# Autodesk Inventor assembly: 垃圾桶
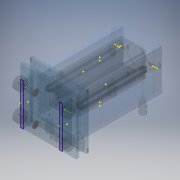
[picture p0: Inventor's stored thumbnail of the model, 180x180]
Saved by Autodesk Inventor 2017 (Build 210142000, 142)
## iProperties
Part Number: 垃圾桶
Material: 常规
Document SubType Name: Assembly
Designer: PANDA
Author: PANDA
## Documents named in this file (22)
- D:\PANDA\Study\VG100\P2\草图\垃圾桶.iam
- D:\PANDA\Study\VG100\P2\草图\垃圾桶正版.ipt
- D:\PANDA\Study\VG100\P2\草图\垃圾桶侧板.ipt
- D:\PANDA\Study\VG100\P2\草图\垃圾桶底板.ipt
- D:\PANDA\Study\VG100\P2\草图\圆柱.ipt
- D:\PANDA\Study\VG100\P2\草图\马达安装板.ipt
- D:\PANDA\Study\VG100\P2\草图\轮子.ipt
- D:\PANDA\Study\VG100\P2\草图\马达.ipt
- D:\PANDA\Study\VG100\P2\草图\红外.ipt
- D:\PANDA\Study\VG100\P2\草图\红外测距.ipt
- D:\PANDA\Study\VG100\P2\草图\姿态传感器.ipt
- D:\PANDA\Study\VG100\P2\草图\激光传感器.ipt
- D:\PANDA\Study\VG100\P2\草图\长轴.ipt
- D:\PANDA\Study\VG100\P2\草图\皮带轮.ipt
- D:\PANDA\Study\VG100\P2\草图\皮带.ipt
- D:\PANDA\Study\VG100\P2\草图\升降板.ipt
- D:\PANDA\Study\VG100\P2\草图\内层升降板.ipt
- D:\PANDA\Study\VG100\P2\草图\内层正板.ipt
- D:\PANDA\Study\VG100\P2\草图\内层侧板.ipt
- D:\PANDA\Study\VG100\P2\草图\推杆电机.ipt
- D:\PANDA\Study\VG100\P2\草图\打包支架.ipt
- D:\PANDA\Study\VG100\P2\草图\压缩杆.ipt
## Components (59 placed, 21 different names)
1. 垃圾桶正版:1 — 旋转:3, 旋转:7, 旋转:8, 旋转:14
2. 垃圾桶侧板:2 — 旋转:3, 旋转:4, 旋转:5, 旋转:13, 刚性:22
3. 垃圾桶正版:2 — 旋转:4, 旋转:5, 旋转:6, 旋转:11, 旋转:32, 旋转:33, 旋转:49, 旋转:50
4. 垃圾桶侧板:3 — 旋转:6, 旋转:7, 旋转:12, 旋转:58
5. 垃圾桶底板:1 — 旋转:8, 旋转:9, 旋转:10, 旋转:15, 旋转:16, 刚性:2, 刚性:3, 刚性:4, 刚性:5, 刚性:21
6. 圆柱:1 — 旋转:9
7. 圆柱:2 — 旋转:10, 旋转:23
8. 圆柱:3 — 旋转:12, 旋转:19
9. 圆柱:4 — 旋转:11
10. 圆柱:5 — 旋转:15
11. 圆柱:6 — 旋转:16, 旋转:17, 旋转:18
12. 圆柱:7 — 旋转:14
13. 圆柱:8 — 旋转:13, 旋转:22
14. 垃圾桶底板:2 — 旋转:17, 刚性:1
15. 马达安装板:1 — 旋转:18, 旋转:19, 旋转:20, 旋转:21
16. 轮子:1 — 旋转:21, 旋转:29
17. 轮子:2 — 旋转:20, 旋转:28
18. 马达安装板:2 — 旋转:22, 旋转:23, 旋转:24, 旋转:25
19. 轮子:3 — 旋转:25, 旋转:27
20. 轮子:4 — 旋转:24, 旋转:26
21. 马达:1 — 旋转:26
22. 马达:2 — 旋转:27
23. 马达:3 — 旋转:28
24. 马达:4 — 旋转:29
25. 红外:1 — 刚性:1
26. 红外测距:1 — 刚性:2
27. 红外测距:2 — 刚性:3
28. 红外测距:3 — 刚性:5
29. 红外测距:4 — 刚性:4
30. 马达:5 — 旋转:33, 旋转:39
31. 马达:7 — 旋转:32, 旋转:36
32. 长轴:2 — 旋转:36, 刚性:8
33. 皮带轮:2 — 刚性:8, 旋转:54
34. 长轴:5 — 旋转:39, 刚性:10
35. 皮带轮:8 — 刚性:10, 旋转:56
36. 升降板:1
37. 升降板:2 — 刚性:17
38. 内层升降板:1 — 刚性:17, 旋转:44, 旋转:45, 旋转:46, 旋转:47, 旋转:48
39. 内层正板:1 — 旋转:44, 旋转:57
40. 内层正板:2 — 旋转:45, 刚性:20
41. 内层侧板:1 — 旋转:46
42. 内层侧板:2 — 旋转:47, 旋转:48
43. 马达:9 — 旋转:49, 旋转:51
44. 长轴:6 — 旋转:52, 刚性:18
45. 长轴:7 — 旋转:51, 刚性:19
46. 马达:10 — 旋转:50, 旋转:52
47. 皮带轮:9 — 刚性:19, 旋转:53
48. 皮带轮:10 — 刚性:18, 旋转:55
49. 皮带:1 — 旋转:53, 旋转:54
50. 皮带:2 — 旋转:55, 旋转:56
51. 激光传感器:3 — 刚性:20
52. 激光传感器:4 — 旋转:57
53. 姿态传感器:1 — 刚性:21
54. 推杆电机:1 — 旋转:58, 旋转:60
55. 打包支架:1 — 旋转:59, 旋转:62
56. 打包支架:2 — 旋转:60, 旋转:61
57. 推杆电机:2 — 刚性:22, 旋转:59
58. 压缩杆:1 — 旋转:61
59. 压缩杆:2 — 旋转:62
## Relationships (63: RevoluteJoint 50, WeldJoint 13)
- 旋转:3 [RevoluteJoint]: 垃圾桶正版:1 ↔ 垃圾桶侧板:2
- 旋转:4 [RevoluteJoint]: 垃圾桶侧板:2 ↔ 垃圾桶正版:2
- 旋转:5 [RevoluteJoint]: 垃圾桶侧板:2 ↔ 垃圾桶正版:2
- 旋转:6 [RevoluteJoint]: 垃圾桶正版:2 ↔ 垃圾桶侧板:3
- 旋转:7 [RevoluteJoint]: 垃圾桶正版:1 ↔ 垃圾桶侧板:3
- 旋转:8 [RevoluteJoint]: 垃圾桶正版:1 ↔ 垃圾桶底板:1
- 旋转:9 [RevoluteJoint]: 垃圾桶底板:1 ↔ 圆柱:1
- 旋转:10 [RevoluteJoint]: 垃圾桶底板:1 ↔ 圆柱:2
- 旋转:11 [RevoluteJoint]: 垃圾桶正版:2 ↔ 圆柱:4
- 旋转:12 [RevoluteJoint]: 垃圾桶侧板:3 ↔ 圆柱:3
- 旋转:13 [RevoluteJoint]: 垃圾桶侧板:2 ↔ 圆柱:8
- 旋转:14 [RevoluteJoint]: 垃圾桶正版:1 ↔ 圆柱:7
- 旋转:15 [RevoluteJoint]: 垃圾桶底板:1 ↔ 圆柱:5
- 旋转:16 [RevoluteJoint]: 垃圾桶底板:1 ↔ 圆柱:6
- 旋转:17 [RevoluteJoint]: 圆柱:6 ↔ 垃圾桶底板:2
- 旋转:18 [RevoluteJoint]: 圆柱:6 ↔ 马达安装板:1
- 旋转:19 [RevoluteJoint]: 圆柱:3 ↔ 马达安装板:1
- 旋转:20 [RevoluteJoint]: 马达安装板:1 ↔ 轮子:2
- 旋转:21 [RevoluteJoint]: 马达安装板:1 ↔ 轮子:1
- 旋转:22 [RevoluteJoint]: 圆柱:8 ↔ 马达安装板:2
- 旋转:23 [RevoluteJoint]: 圆柱:2 ↔ 马达安装板:2
- 旋转:24 [RevoluteJoint]: 马达安装板:2 ↔ 轮子:4
- 旋转:25 [RevoluteJoint]: 马达安装板:2 ↔ 轮子:3
- 旋转:26 [RevoluteJoint]: 轮子:4 ↔ 马达:1
- 旋转:27 [RevoluteJoint]: 轮子:3 ↔ 马达:2
- 旋转:28 [RevoluteJoint]: 轮子:2 ↔ 马达:3
- 旋转:29 [RevoluteJoint]: 轮子:1 ↔ 马达:4
- 刚性:1 [WeldJoint]: 垃圾桶底板:2 ↔ 红外:1
- 刚性:2 [WeldJoint]: 垃圾桶底板:1 ↔ 红外测距:1
- 刚性:3 [WeldJoint]: 垃圾桶底板:1 ↔ 红外测距:2
- 刚性:4 [WeldJoint]: 垃圾桶底板:1 ↔ 红外测距:4
- 刚性:5 [WeldJoint]: 垃圾桶底板:1 ↔ 红外测距:3
- 旋转:32 [RevoluteJoint]: 垃圾桶正版:2 ↔ 马达:7
- 旋转:33 [RevoluteJoint]: 垃圾桶正版:2 ↔ 马达:5
- 旋转:36 [RevoluteJoint]: 马达:7 ↔ 长轴:2
- 刚性:8 [WeldJoint]: 长轴:2 ↔ 皮带轮:2
- 旋转:39 [RevoluteJoint]: 马达:5 ↔ 长轴:5
- 刚性:10 [WeldJoint]: 长轴:5 ↔ 皮带轮:8
- 刚性:17 [WeldJoint]: 升降板:2 ↔ 内层升降板:1
- 旋转:44 [RevoluteJoint]: 内层升降板:1 ↔ 内层正板:1
- 旋转:45 [RevoluteJoint]: 内层升降板:1 ↔ 内层正板:2
- 旋转:46 [RevoluteJoint]: 内层升降板:1 ↔ 内层侧板:1
- 旋转:47 [RevoluteJoint]: 内层升降板:1 ↔ 内层侧板:2
- 旋转:48 [RevoluteJoint]: 内层升降板:1 ↔ 内层侧板:2
- 旋转:49 [RevoluteJoint]: 垃圾桶正版:2 ↔ 马达:9
- 旋转:50 [RevoluteJoint]: 垃圾桶正版:2 ↔ 马达:10
- 旋转:51 [RevoluteJoint]: 马达:9 ↔ 长轴:7
- 旋转:52 [RevoluteJoint]: 长轴:6 ↔ 马达:10
- 刚性:18 [WeldJoint]: 长轴:6 ↔ 皮带轮:10
- 刚性:19 [WeldJoint]: 长轴:7 ↔ 皮带轮:9
- 旋转:53 [RevoluteJoint]: 皮带轮:9 ↔ 皮带:1
- 旋转:54 [RevoluteJoint]: 皮带轮:2 ↔ 皮带:1
- 旋转:55 [RevoluteJoint]: 皮带轮:10 ↔ 皮带:2
- 旋转:56 [RevoluteJoint]: 皮带轮:8 ↔ 皮带:2
- 刚性:20 [WeldJoint]: 内层正板:2 ↔ 激光传感器:3
- 旋转:57 [RevoluteJoint]: 内层正板:1 ↔ 激光传感器:4
- 刚性:21 [WeldJoint]: 垃圾桶底板:1 ↔ 姿态传感器:1
- 旋转:58 [RevoluteJoint]: 垃圾桶侧板:3 ↔ 推杆电机:1
- 刚性:22 [WeldJoint]: 垃圾桶侧板:2 ↔ 推杆电机:2
- 旋转:59 [RevoluteJoint]: 打包支架:1 ↔ 推杆电机:2
- 旋转:60 [RevoluteJoint]: 推杆电机:1 ↔ 打包支架:2
- 旋转:61 [RevoluteJoint]: 打包支架:2 ↔ 压缩杆:1
- 旋转:62 [RevoluteJoint]: 打包支架:1 ↔ 压缩杆:2
